# Autodesk Inventor assembly: Assembly_Fischer_speedmax_3D
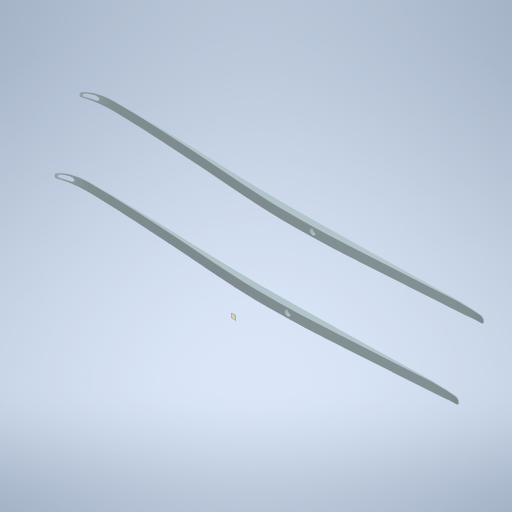
[picture p0: Inventor's stored thumbnail of the model, 512x512]
Saved by Autodesk Inventor 2024 (Build 280153000, 153)
## iProperties
Created: 2023-10-23
Part Number: Assembly_Fischer_speedmax_3D
Document SubType Name: Assembly
Designer: tinas
Sending System: Autodesk Inventor 2024
Preprocessor: ST-DEVELOPER v19.2
Title: Skii.stp
Author: tinas
## Documents named in this file (3)
- C:\Users\tinas\OneDrive\Desktop\SpeedRiding\SpeedRiding\CAD\Skii\Skii.iam
- C:\Users\tinas\OneDrive\Desktop\SpeedRiding\SpeedRiding\CAD\Skii\Skida_gusaxe-7.ipt
- C:\Users\tinas\OneDrive\Desktop\SpeedRiding\SpeedRiding\CAD\Skii\SKC\SKC.iam
## Components (2 placed, 2 different names)
1. Skida_gusaxe-7_1018 — Flush:1
2. SKC:1 [sub-assembly]
## Relationships (1: Flush 1)
- Flush:1: Skida_gusaxe-7_1018
